# Autodesk Inventor assembly: FullLegAssembly
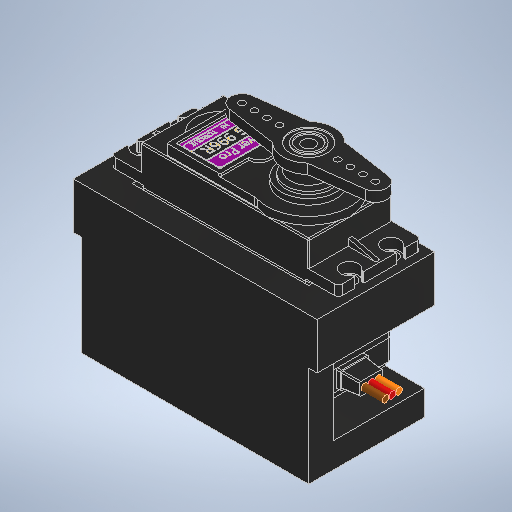
[picture p0: Inventor's stored thumbnail of the model, 512x512]
Saved by Autodesk Inventor 2025 (Build 290162000, 162)
## iProperties
Created: 2024-09-10
Part Number: FullLegAssembly
Document SubType Name: Assembly
Designer: omiye
Author: omiye
## Documents named in this file (4)
- C:\Users\7008661\Downloads\hexapod\legModels\FullLegAssembly.iam
- C:\Users\7008661\Downloads\hexapod\legModels\MG996RServo.ipt
- C:\Users\7008661\Downloads\hexapod\legModels\MG996RServoHolder.ipt
- C:\Users\7008661\Downloads\hexapod\legModels\straightServoHorn.ipt
## Components (3 placed, 3 different names)
1. MG996RServo:1 — Mate:1, Mate:2, Mate:5, Mate:6, Mate:9, Mate:10, Mate:11, Mate:12
2. MG996RServoHolder:1 — Mate:1, Mate:2, Mate:9, Mate:10, Mate:11, Mate:12
3. straightServoHorn:1 — Mate:5, Mate:6
## Relationships (8: Mate 8)
- Mate:1: MG996RServo:1 ↔ MG996RServoHolder:1
- Mate:2: MG996RServo:1 ↔ MG996RServoHolder:1
- Mate:5: MG996RServo:1 ↔ straightServoHorn:1
- Mate:6: MG996RServo:1 ↔ straightServoHorn:1
- Mate:9: MG996RServo:1 ↔ MG996RServoHolder:1
- Mate:10: MG996RServo:1 ↔ MG996RServoHolder:1
- Mate:11: MG996RServo:1 ↔ MG996RServoHolder:1
- Mate:12: MG996RServo:1 ↔ MG996RServoHolder:1
